# Autodesk Inventor assembly: ybeltsupport
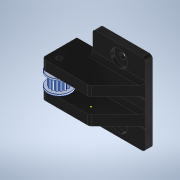
[picture p0: Inventor's stored thumbnail of the model, 180x180]
Saved by Autodesk Inventor 2020.2 (Build 242310000, 310)
## iProperties
Created: 2020-08-06
Part Number: ybeltsupport
Document SubType Name: Assembly
Designer: JK
Author: JK
## Documents named in this file (3)
- C:\Users\JK\Documents\Inventor\Anet Upgrade\ybeltsupport.iam
- C:\Users\JK\Documents\Inventor\Anet Upgrade\GT2 Timing Idler Pulley, Configurable, 16T W6 B3 With T.iam
- C:\Users\JK\Documents\Inventor\Anet Upgrade\pulleysupport.ipt
## Components (2 placed, 2 different names)
1. GT2 Timing Idler Pulley, Configurable, 16T W6 B3 With T:1 [sub-assembly] — Mate:1, Mate:2
2. pulleysupport:1 — Mate:1, Mate:2
## Relationships (2: Mate 2)
- Mate:1: GT2 Timing Idler Pulley, Configurable, 16T W6 B3 With T:1 ↔ pulleysupport:1
- Mate:2 (0.25 mm): GT2 Timing Idler Pulley, Configurable, 16T W6 B3 With T:1 ↔ pulleysupport:1
